# Autodesk Inventor assembly: BG_Schiffschraube
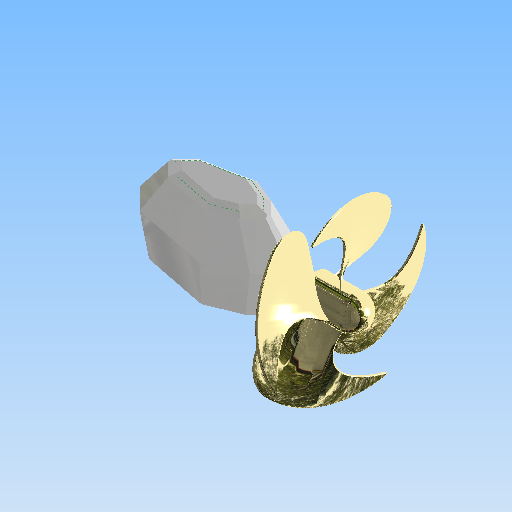
[picture p0: Inventor's stored thumbnail of the model, 512x512]
Saved by Autodesk Inventor 2024.4 (Build 284460000, 460)
## iProperties
Created: 2026-01-21
Part Number: BG_Schiffschraube
Document SubType Name: Assembly
Designer: windows-desktop
Mass: 1421.56 g
Surface Area: 3067.46 cm^2
Volume: 788.261 cm^3
Density: 1.80342 g/cm^3
Author: windows-desktop
## Documents named in this file (9)
- C:\Users\windows-desktop\Desktop\Studium\Konstruktion\VaultWorkspace\Daten\I60-Konstruktion\I60-Gruppe-4\Bluhm\Daten\I60-Konstruktion\I60-Gruppe-4\Bluhm\Antrieb\BG_Schiffschraube.iam
- C:\Users\windows-desktop\Desktop\Studium\Konstruktion\VaultWorkspace\Daten\I60-Konstruktion\I60-Gruppe-4\Bluhm\Daten\I60-Konstruktion\I60-Gruppe-4\Bluhm\Antrieb\Schrauben_Block.ipt
- C:\Users\windows-desktop\Desktop\Studium\Konstruktion\VaultWorkspace\Daten\I60-Konstruktion\I60-Gruppe-4\Bluhm\Daten\I60-Konstruktion\I60-Gruppe-4\Bluhm\Antrieb\Propeller_groß.ipt
- C:\Users\windows-desktop\Desktop\Studium\Konstruktion\VaultWorkspace\Daten\I60-Konstruktion\I60-Gruppe-4\Bluhm\Normteile\de-DE\DIN 3760 A\DIN 3760 - A - 30 x 40 x 7 - NBR.ipt
- C:\Users\windows-desktop\Desktop\Studium\Konstruktion\VaultWorkspace\Daten\I60-Konstruktion\I60-Gruppe-4\Bluhm\Normteile\de-DE\DIN 625 SKF(3)\DIN 625 SKF - SKF (61806-RZ).ipt
- C:\Users\windows-desktop\Desktop\Studium\Konstruktion\VaultWorkspace\Daten\I60-Konstruktion\I60-Gruppe-4\Bluhm\Daten\I60-Konstruktion\I60-Gruppe-4\Bluhm\Antrieb\Wellennut_Antrieb_Schrauben_Block.ipt
- C:\Users\windows-desktop\Desktop\Studium\Konstruktion\VaultWorkspace\Daten\I60-Konstruktion\I60-Gruppe-4\Bluhm\Daten\I60-Konstruktion\I60-Gruppe-4\Bluhm\Antrieb\Wellennut_Antrieb_Propeller.ipt
- C:\Users\windows-desktop\Desktop\Studium\Konstruktion\VaultWorkspace\Daten\I60-Konstruktion\I60-Gruppe-4\Bluhm\Daten\I60-Konstruktion\I60-Gruppe-4\Bluhm\Antrieb\Kegelrad01.ipt
- C:\Users\windows-desktop\Desktop\Studium\Konstruktion\VaultWorkspace\Daten\I60-Konstruktion\I60-Gruppe-4\Bluhm\Daten\I60-Konstruktion\I60-Gruppe-4\Bluhm\Antrieb\Welle_Schraube.ipt
## Components (8 placed, 8 different names)
1. Schrauben_Block:1 — Einfügen:2, Einfügen:3
2. DIN 3760 A A - 30 x 40 x 7 - NBR:1 — Einfügen:2
3. DIN 625 SKF- mit Dichtung mit niedriger Reibung, einseitig abgedichtet SKF (61806-RZ):1 — Einfügen:3, Einfügen:4
4. Propeller_groß:3 — Fluchtend:3, Passend:5, Passend:8
5. Welle_Schraube:1 — Fluchtend:1, Passend:1, Passend:2, Fluchtend:2, Passend:3, Passend:4
6. Wellennut_Antrieb_Propeller:1 — Fluchtend:2, Passend:3, Passend:4, Fluchtend:3, Passend:5, Passend:8
7. Wellennut_Antrieb_Schrauben_Block:1 — Fluchtend:1, Passend:1, Passend:2, Fluchtend:4, Passend:6, Passend:7
8. Kegelrad1:1 — Fluchtend:4, Passend:6, Passend:7, Einfügen:4
## Relationships (15: Mate 8, Flush 4, Insert 3)
- Einfügen:2 [Insert]: Schrauben_Block:1 ↔ DIN 3760 A A - 30 x 40 x 7 - NBR:1
- Einfügen:3 [Insert]: Schrauben_Block:1 ↔ DIN 625 SKF- mit Dichtung mit niedriger Reibung, einseitig abgedichtet SKF (61806-RZ):1
- Fluchtend:1 [Flush]: Welle_Schraube:1 ↔ Wellennut_Antrieb_Schrauben_Block:1
- Passend:1 [Mate]: Welle_Schraube:1 ↔ Wellennut_Antrieb_Schrauben_Block:1
- Passend:2 [Mate]: Welle_Schraube:1 ↔ Wellennut_Antrieb_Schrauben_Block:1
- Fluchtend:2 [Flush]: Welle_Schraube:1 ↔ Wellennut_Antrieb_Propeller:1
- Passend:3 [Mate]: Welle_Schraube:1 ↔ Wellennut_Antrieb_Propeller:1
- Passend:4 [Mate]: Welle_Schraube:1 ↔ Wellennut_Antrieb_Propeller:1
- Fluchtend:3 [Flush]: Propeller_groß:3 ↔ Wellennut_Antrieb_Propeller:1
- Passend:5 [Mate]: Propeller_groß:3 ↔ Wellennut_Antrieb_Propeller:1
- Fluchtend:4 [Flush]: Wellennut_Antrieb_Schrauben_Block:1 ↔ Kegelrad1:1
- Passend:6 [Mate]: Wellennut_Antrieb_Schrauben_Block:1 ↔ Kegelrad1:1
- Passend:7 [Mate]: Wellennut_Antrieb_Schrauben_Block:1 ↔ Kegelrad1:1
- Passend:8 [Mate]: Propeller_groß:3 ↔ Wellennut_Antrieb_Propeller:1
- Einfügen:4 [Insert] (6 mm): DIN 625 SKF- mit Dichtung mit niedriger Reibung, einseitig abgedichtet SKF (61806-RZ):1 ↔ Kegelrad1:1
